# Autodesk Inventor assembly: keypad and cover
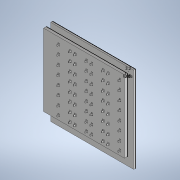
[picture p0: Inventor's stored thumbnail of the model, 180x180]
Saved by Autodesk Inventor 2022 (Build 260153000, 153)
## iProperties
Created: 2022-05-25
Part Number: keypad and cover
Document SubType Name: Assembly
Designer: alecw
Author: alecw
## Documents named in this file (3)
- C:\aw_od\OneDrive\Desktop\keypad and cover.iam
- C:\aw_gd\Coding and Projects\smart home\smart-deadbolt\3D Modelling\4x4 keypad flexible cover v2.ipt
- C:\aw_gd\Coding and Projects\smart home\smart-deadbolt\3D Modelling\4x4 keypad model.ipt
## Components (2 placed, 2 different names)
1. 4x4 keypad flexible cover v2:1 — Mate:2, Mate:3, Mate:4
2. 4x4 keypad model:1 — Mate:2, Mate:3, Mate:4
## Relationships (3: Mate 3)
- Mate:2 (0.354 mm): 4x4 keypad flexible cover v2:1 ↔ 4x4 keypad model:1
- Mate:3 (0.354 mm): 4x4 keypad flexible cover v2:1 ↔ 4x4 keypad model:1
- Mate:4: 4x4 keypad flexible cover v2:1 ↔ 4x4 keypad model:1
